# Autodesk Inventor assembly: bepf
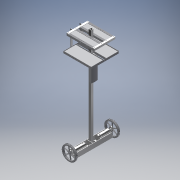
[picture p0: Inventor's stored thumbnail of the model, 180x180]
Saved by Autodesk Inventor 2017 (Build 210142000, 142)
## iProperties
Part Number: bepf
Material: Ogólny
Document SubType Name: Assembly
Designer: gagato
Author: gagato
## Documents named in this file (5)
- C:\Users\gagato\Documents\bepf\Inventor\bepf.iam
- C:\Users\gagato\Documents\bepf\Inventor\bepf_podwozie.iam
- C:\Users\gagato\Documents\bepf\Inventor\bepf_platforma.iam
- C:\Users\gagato\Documents\bepf\Inventor\bepf_platforma_wspornik_poziomy.ipt
- C:\Users\gagato\Documents\bepf\Inventor\bepf_bateria_lipo.ipt
## Components (5 placed, 4 different names)
1. bepf_podwozie:1 [sub-assembly] — Zestawiający:1, Zestawiający:2, Zestawiający:3, Zestawiający:4, Zestawiający:5, Zestawiający:6, Zestawiający:8, Zestawiający:9, Zestawiający:11, Równoległy:1
2. bepf_platforma:1 [sub-assembly] — Zestawiający:2, Zestawiający:3, Zestawiający:4, Zestawiający:7, Zestawiający:10
3. bepf_platforma_wspornik_poziomy:1 — Zestawiający:5, Zestawiający:6, Zestawiający:7, Zestawiający:12
4. bepf_platforma_wspornik_poziomy:2 — Zestawiający:8, Zestawiający:9, Zestawiający:10
5. bepf_bateria_lipo:1 — Zestawiający:11, Zestawiający:12, Równoległy:1
## Relationships (13: Mate 12, Flush 1)
- Zestawiający:1 [Mate]: bepf_podwozie:1
- Zestawiający:2 [Mate]: bepf_podwozie:1 ↔ bepf_platforma:1
- Zestawiający:3 [Mate]: bepf_podwozie:1 ↔ bepf_platforma:1
- Zestawiający:4 [Mate]: bepf_podwozie:1 ↔ bepf_platforma:1
- Zestawiający:5 [Mate]: bepf_podwozie:1 ↔ bepf_platforma_wspornik_poziomy:1
- Zestawiający:6 [Mate]: bepf_podwozie:1 ↔ bepf_platforma_wspornik_poziomy:1
- Zestawiający:7 [Mate]: bepf_platforma:1 ↔ bepf_platforma_wspornik_poziomy:1
- Zestawiający:8 [Mate]: bepf_podwozie:1 ↔ bepf_platforma_wspornik_poziomy:2
- Zestawiający:9 [Mate]: bepf_podwozie:1 ↔ bepf_platforma_wspornik_poziomy:2
- Zestawiający:10 [Mate]: bepf_platforma:1 ↔ bepf_platforma_wspornik_poziomy:2
- Zestawiający:11 [Mate]: bepf_podwozie:1 ↔ bepf_bateria_lipo:1
- Zestawiający:12 [Mate]: bepf_platforma_wspornik_poziomy:1 ↔ bepf_bateria_lipo:1
- Równoległy:1 [Flush] (-12.5 mm): bepf_podwozie:1 ↔ bepf_bateria_lipo:1
